# Autodesk Inventor assembly: Battery_Slide
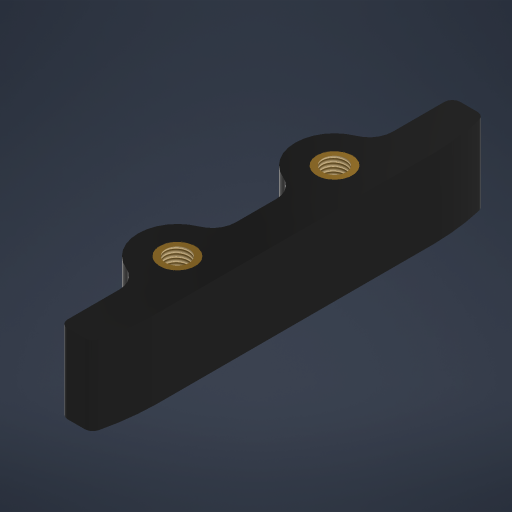
[picture p0: Inventor's stored thumbnail of the model, 512x512]
Saved by Autodesk Inventor 2024 (Build 280153000, 153)
## iProperties
Created: 2023-06-20
Part Number: Battery_Slide
Document SubType Name: Assembly
Designer: dzw04
Author: dzw04
## Documents named in this file (3)
- C:\Users\dzw04\Saxion\Mechatronica Lectoraat LMECH LED - Database ARG\Component_Database\SAR\01. CAD\01. 3D_Drawing\02. Sub_Assemblies\Battery_Slide.iam
- C:\Users\dzw04\Saxion\Mechatronica Lectoraat LMECH LED - Database ARG\Component_Database\SAR\01. CAD\01. 3D_Drawing\01. Parts\Battery_Slide.ipt
- C:\Users\dzw04\Saxion\Mechatronica Lectoraat LMECH LED - Database ARG\Component_Database\SAR\01. CAD\01. 3D_Drawing\01. Parts\Threaded_Insert_M3x4.ipt
## Components (5 placed, 2 different names)
1. Battery_Slide:1 — Flush:1, Flush:2, Flush:3, Flush:4, Mate:1, Mate:2, Mate:3, Mate:4
2. Threaded_Insert_M3x4:1 — Flush:1, Mate:4
3. Threaded_Insert_M3x4:2 — Flush:2, Mate:3
4. Threaded_Insert_M3x4:3 — Flush:3, Mate:2
5. Threaded_Insert_M3x4:4 — Flush:4, Mate:1
## Relationships (8: Flush 4, Mate 4)
- Flush:1: Battery_Slide:1 ↔ Threaded_Insert_M3x4:1
- Flush:2: Battery_Slide:1 ↔ Threaded_Insert_M3x4:2
- Flush:3: Battery_Slide:1 ↔ Threaded_Insert_M3x4:3
- Flush:4: Battery_Slide:1 ↔ Threaded_Insert_M3x4:4
- Mate:1: Battery_Slide:1 ↔ Threaded_Insert_M3x4:4
- Mate:2: Battery_Slide:1 ↔ Threaded_Insert_M3x4:3
- Mate:3: Battery_Slide:1 ↔ Threaded_Insert_M3x4:2
- Mate:4: Battery_Slide:1 ↔ Threaded_Insert_M3x4:1
